# Autodesk Inventor assembly: Shooter Oct10
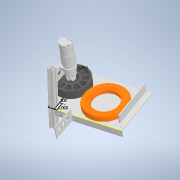
[picture p0: Inventor's stored thumbnail of the model, 180x180]
Saved by Autodesk Inventor 2020.3 (Build 243373010, 373A)
## iProperties
Created: 2020-10-10
Part Number: Shooter Oct10
Document SubType Name: Assembly
Designer: Owner
Author: Owner
## Documents named in this file (10)
- C:\Users\Owner\Documents\GitHub\CAD-2021-Ultimate_Goal\Shooter\Shooter Oct10.iam
- C:\Users\Owner\Documents\GitHub\CAD-2021-Ultimate_Goal\ServoCity\7in-Xrail.ipt
- C:\Users\Owner\Documents\GitHub\CAD-2021-Ultimate_Goal\ServoCity\555176 assembly.ipt
- C:\Users\Owner\Documents\GitHub\CAD-2021-Ultimate_Goal\ServoCity\585720.ipt
- C:\Users\Owner\Documents\GitHub\CAD-2021-Ultimate_Goal\GoBilda\5202-0002-0003 part.ipt
- C:\Users\Owner\Documents\GitHub\CAD-2021-Ultimate_Goal\Shooter\Shooter plate but for an xrail.ipt
- C:\Users\Owner\Documents\GitHub\CAD-2021-Ultimate_Goal\AndyMark\am-3563 4IN 8mm Round Compliant Wheel REV2.ipt
- C:\Users\Owner\Documents\GitHub\CAD-2021-Ultimate_Goal\ServoCity\545456.ipt
- C:\Users\Owner\Documents\GitHub\CAD-2021-Ultimate_Goal\ServoCity\545636 assembly.ipt
- C:\Users\Owner\Documents\GitHub\CAD-2021-Ultimate_Goal\AndyMark\am-4300 Ring.ipt
## Components (11 placed, 9 different names)
1. 7in-Xrail:1 — Mate:5, Mate:12, Mate:25
2. 585720:1 — Mate:6, Mate:7, Mate:8, Mate:25
3. 7in-Xrail:2 — Mate:5, Mate:10, Mate:11
4. 5202-0002-0003 part:1 — Mate:9, Mate:14, Mate:15, Mate:21
5. 555176 assembly:1 — Mate:6, Mate:7, Mate:8, Mate:9, Mate:21
6. Shooter plate but for an xrail:1 — Mate:10, Mate:11, Mate:12, Mate:24
7. am-3563 4IN 8mm Round Compliant Wheel REV2:1 — Mate:22, Mate:23
8. 545456:1 — Mate:13, Mate:16, Mate:17, Mate:22, Mate:23
9. 545636 assembly:1 — Mate:13, Mate:14, Mate:15, Mate:16, Mate:17
10. am-4300 Ring:1 — Mate:24
11. 585720:2
## Relationships (18: Mate 18)
- Mate:5: 7in-Xrail:1 ↔ 7in-Xrail:2
- Mate:6: 585720:1 ↔ 555176 assembly:1
- Mate:7: 585720:1 ↔ 555176 assembly:1
- Mate:8: 585720:1 ↔ 555176 assembly:1
- Mate:9: 5202-0002-0003 part:1 ↔ 555176 assembly:1
- Mate:10: 7in-Xrail:2 ↔ Shooter plate but for an xrail:1
- Mate:11: 7in-Xrail:2 ↔ Shooter plate but for an xrail:1
- Mate:12: 7in-Xrail:1 ↔ Shooter plate but for an xrail:1
- Mate:13: 545456:1 ↔ 545636 assembly:1
- Mate:14: 5202-0002-0003 part:1 ↔ 545636 assembly:1
- Mate:15: 5202-0002-0003 part:1 ↔ 545636 assembly:1
- Mate:16: 545456:1 ↔ 545636 assembly:1
- Mate:17: 545456:1 ↔ 545636 assembly:1
- Mate:21: 5202-0002-0003 part:1 ↔ 555176 assembly:1
- Mate:22: am-3563 4IN 8mm Round Compliant Wheel REV2:1 ↔ 545456:1
- Mate:23: am-3563 4IN 8mm Round Compliant Wheel REV2:1 ↔ 545456:1
- Mate:24: Shooter plate but for an xrail:1 ↔ am-4300 Ring:1
- Mate:25: 7in-Xrail:1 ↔ 585720:1
